# Autodesk Inventor assembly: 51111
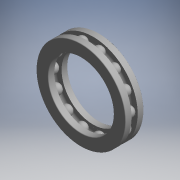
[picture p0: Inventor's stored thumbnail of the model, 180x180]
Saved by Autodesk Inventor 2023 (Build 270158000, 158)
## iProperties
Part Number: 51111
Catalog Web Link: www.cadenas.de
Description: Single Direction Type-
Vendor: NTN
Document SubType Name: Assembly
Designer: partserver
Manufacturer: NTN
Mass: 26.0815 g
Surface Area: 175.483 cm^2
Volume: 26.0815 cm^3
Density: 1 g/cm^3
Category: PARTsolutions
Company: NTN
PSOL_IDENT_0: {$CADENAS_DATA\23d-libs\ntn\ball_roller_bearings\thrust_b\tb_sdt_asmtab.prj},182 {VTYP=3D},{STYP=ASS
PSOL_IDENT_1: TAB},{NB=51111},{LINA=51111},{NN=Single Direction Type},{DATE=21.12.2021 04:23:12},{GEOMDATE=17.04.2
PSOL_IDENT_2: 020 05:29:34},{VERSION=},{LINEID=11140},{WBVAR=},{WBNUMERIC=}  {NB=51111},{LINA=51111},{KT=DUMMY},{I
PSOL_IDENT_3: DNR=},{SD=55},{D=78},{T=16},{R=0.6},{ORDER=51111},{CA=35},{COA=93},{CU=4.2},{CAF=3 550},{COAF=9 500}
PSOL_IDENT_4: ,{NG=2 800},{NO=4 000},{D1=78},{SD1=57},{MASS=0.23},{DA1=69},{DA=64},{RAS=0,6},{X=10.50000},{BN=13.3
PSOL_IDENT_5: 16964},{X1=11.50000},{O=208.81},{T1=5.33333},{T2=5.33333},{RB=4.48000},{PPATH=tb_sdt_asmtpl.prj}
NB: 51111
NN: Single Direction Type
NBSYN: $ORDER.
LINA: 51111
CATALOG: NTN Corporation
SD: 55
D: 78
T: 16
R: 0.6
ORDER: 51111
CA: 35
COA: 93
CU: 4.2
NG: 2 800
NO: 4 000
D1: 78
SD1: 57
MASS: 0.23
SUPPLIER: NTN
ARTICLENO: 51111
BOMINFO: 51111
CREATOR: CADENAS GmbH
Title: 51111
Author: Cadenas PARTsolutions
## Documents named in this file (4)
- C:\Users\adash\OneDrive - Kyushu University\Attachments\ロボコン\catchrobo2022\CAD\Adachi\theta\51111.iam
- C:\Users\adash\OneDrive - Kyushu University\Attachments\ロボコン\catchrobo2022\CAD\Adachi\theta\51111 Housing raceway disc.ipt
- C:\Users\adash\OneDrive - Kyushu University\Attachments\ロボコン\catchrobo2022\CAD\Adachi\theta\51111 Shaft raceway disc.ipt
- C:\Users\adash\OneDrive - Kyushu University\Attachments\ロボコン\catchrobo2022\CAD\Adachi\theta\51111 Ball.ipt
## Components (16 placed, 3 different names)
1. 51111 Housing raceway disc:1 — tb_sdt_hrd_XY@1 <-> tb_sdt_srd_XY@2, tb_sdt_hrd_Z@1 <-> tb_sdt_srd_Z@2, tb_sdt_hrd_YZ@1 <-> tb_sdt_srd_YZ@2
2. 51111 Shaft raceway disc:1 — tb_sdt_hrd_XY@1 <-> tb_sdt_srd_XY@2, tb_sdt_hrd_Z@1 <-> tb_sdt_srd_Z@2, tb_sdt_hrd_YZ@1 <-> tb_sdt_srd_YZ@2, tb_sdt_srd1_1_XY@2 <-> tb_sdt_b_XY@3, tb_sdt_srd1_1_Z@2 <-> tb_sdt_b_Z@3, tb_sdt_srd1_1_YZ@2 <-> tb_sdt_b_YZ@3, tb_sdt_srd1_2_XY@2 <-> tb_sdt_b_XY@4, tb_sdt_srd1_2_Z@2 <-> tb_sdt_b_Z@4, tb_sdt_srd1_2_YZ@2 <-> tb_sdt_b_YZ@4, tb_sdt_srd1_3_XY@2 <-> tb_sdt_b_XY@5, tb_sdt_srd1_3_Z@2 <-> tb_sdt_b_Z@5, tb_sdt_srd1_3_YZ@2 <-> tb_sdt_b_YZ@5, tb_sdt_srd1_4_XY@2 <-> tb_sdt_b_XY@6, tb_sdt_srd1_4_Z@2 <-> tb_sdt_b_Z@6, tb_sdt_srd1_4_YZ@2 <-> tb_sdt_b_YZ@6, tb_sdt_srd1_5_XY@2 <-> tb_sdt_b_XY@7, tb_sdt_srd1_5_Z@2 <-> tb_sdt_b_Z@7, tb_sdt_srd1_5_YZ@2 <-> tb_sdt_b_YZ@7, tb_sdt_srd1_6_XY@2 <-> tb_sdt_b_XY@8, tb_sdt_srd1_6_Z@2 <-> tb_sdt_b_Z@8, tb_sdt_srd1_6_YZ@2 <-> tb_sdt_b_YZ@8, tb_sdt_srd1_7_XY@2 <-> tb_sdt_b_XY@9, tb_sdt_srd1_7_Z@2 <-> tb_sdt_b_Z@9, tb_sdt_srd1_7_YZ@2 <-> tb_sdt_b_YZ@9, tb_sdt_srd1_8_XY@2 <-> tb_sdt_b_XY@10, tb_sdt_srd1_8_Z@2 <-> tb_sdt_b_Z@10, tb_sdt_srd1_8_YZ@2 <-> tb_sdt_b_YZ@10, tb_sdt_srd1_9_XY@2 <-> tb_sdt_b_XY@11, tb_sdt_srd1_9_Z@2 <-> tb_sdt_b_Z@11, tb_sdt_srd1_9_YZ@2 <-> tb_sdt_b_YZ@11, tb_sdt_srd1_10_XY@2 <-> tb_sdt_b_XY@12, tb_sdt_srd1_10_Z@2 <-> tb_sdt_b_Z@12, tb_sdt_srd1_10_YZ@2 <-> tb_sdt_b_YZ@12, tb_sdt_srd1_11_XY@2 <-> tb_sdt_b_XY@13, tb_sdt_srd1_11_Z@2 <-> tb_sdt_b_Z@13, tb_sdt_srd1_11_YZ@2 <-> tb_sdt_b_YZ@13, tb_sdt_srd1_12_XY@2 <-> tb_sdt_b_XY@14, tb_sdt_srd1_12_Z@2 <-> tb_sdt_b_Z@14, tb_sdt_srd1_12_YZ@2 <-> tb_sdt_b_YZ@14, tb_sdt_srd1_13_XY@2 <-> tb_sdt_b_XY@15, tb_sdt_srd1_13_Z@2 <-> tb_sdt_b_Z@15, tb_sdt_srd1_13_YZ@2 <-> tb_sdt_b_YZ@15, tb_sdt_srd1_14_XY@2 <-> tb_sdt_b_XY@16, tb_sdt_srd1_14_Z@2 <-> tb_sdt_b_Z@16, tb_sdt_srd1_14_YZ@2 <-> tb_sdt_b_YZ@16
3. 51111 Ball:1 — tb_sdt_srd1_1_XY@2 <-> tb_sdt_b_XY@3, tb_sdt_srd1_1_Z@2 <-> tb_sdt_b_Z@3, tb_sdt_srd1_1_YZ@2 <-> tb_sdt_b_YZ@3
4. 51111 Ball:2 — tb_sdt_srd1_2_XY@2 <-> tb_sdt_b_XY@4, tb_sdt_srd1_2_Z@2 <-> tb_sdt_b_Z@4, tb_sdt_srd1_2_YZ@2 <-> tb_sdt_b_YZ@4
5. 51111 Ball:3 — tb_sdt_srd1_3_XY@2 <-> tb_sdt_b_XY@5, tb_sdt_srd1_3_Z@2 <-> tb_sdt_b_Z@5, tb_sdt_srd1_3_YZ@2 <-> tb_sdt_b_YZ@5
6. 51111 Ball:4 — tb_sdt_srd1_4_XY@2 <-> tb_sdt_b_XY@6, tb_sdt_srd1_4_Z@2 <-> tb_sdt_b_Z@6, tb_sdt_srd1_4_YZ@2 <-> tb_sdt_b_YZ@6
7. 51111 Ball:5 — tb_sdt_srd1_5_XY@2 <-> tb_sdt_b_XY@7, tb_sdt_srd1_5_Z@2 <-> tb_sdt_b_Z@7, tb_sdt_srd1_5_YZ@2 <-> tb_sdt_b_YZ@7
8. 51111 Ball:6 — tb_sdt_srd1_6_XY@2 <-> tb_sdt_b_XY@8, tb_sdt_srd1_6_Z@2 <-> tb_sdt_b_Z@8, tb_sdt_srd1_6_YZ@2 <-> tb_sdt_b_YZ@8
9. 51111 Ball:7 — tb_sdt_srd1_7_XY@2 <-> tb_sdt_b_XY@9, tb_sdt_srd1_7_Z@2 <-> tb_sdt_b_Z@9, tb_sdt_srd1_7_YZ@2 <-> tb_sdt_b_YZ@9
10. 51111 Ball:8 — tb_sdt_srd1_8_XY@2 <-> tb_sdt_b_XY@10, tb_sdt_srd1_8_Z@2 <-> tb_sdt_b_Z@10, tb_sdt_srd1_8_YZ@2 <-> tb_sdt_b_YZ@10
11. 51111 Ball:9 — tb_sdt_srd1_9_XY@2 <-> tb_sdt_b_XY@11, tb_sdt_srd1_9_Z@2 <-> tb_sdt_b_Z@11, tb_sdt_srd1_9_YZ@2 <-> tb_sdt_b_YZ@11
12. 51111 Ball:10 — tb_sdt_srd1_10_XY@2 <-> tb_sdt_b_XY@12, tb_sdt_srd1_10_Z@2 <-> tb_sdt_b_Z@12, tb_sdt_srd1_10_YZ@2 <-> tb_sdt_b_YZ@12
13. 51111 Ball:11 — tb_sdt_srd1_11_XY@2 <-> tb_sdt_b_XY@13, tb_sdt_srd1_11_Z@2 <-> tb_sdt_b_Z@13, tb_sdt_srd1_11_YZ@2 <-> tb_sdt_b_YZ@13
14. 51111 Ball:12 — tb_sdt_srd1_12_XY@2 <-> tb_sdt_b_XY@14, tb_sdt_srd1_12_Z@2 <-> tb_sdt_b_Z@14, tb_sdt_srd1_12_YZ@2 <-> tb_sdt_b_YZ@14
15. 51111 Ball:13 — tb_sdt_srd1_13_XY@2 <-> tb_sdt_b_XY@15, tb_sdt_srd1_13_Z@2 <-> tb_sdt_b_Z@15, tb_sdt_srd1_13_YZ@2 <-> tb_sdt_b_YZ@15
16. 51111 Ball:14 — tb_sdt_srd1_14_XY@2 <-> tb_sdt_b_XY@16, tb_sdt_srd1_14_Z@2 <-> tb_sdt_b_Z@16, tb_sdt_srd1_14_YZ@2 <-> tb_sdt_b_YZ@16
## Relationships (45: Mate 29, Angle 15, Flush 1)
- tb_sdt_hrd_XY@1 <-> tb_sdt_srd_XY@2 [Flush]: 51111 Housing raceway disc:1 ↔ 51111 Shaft raceway disc:1
- tb_sdt_hrd_Z@1 <-> tb_sdt_srd_Z@2 [Mate]: 51111 Housing raceway disc:1 ↔ 51111 Shaft raceway disc:1
- tb_sdt_hrd_YZ@1 <-> tb_sdt_srd_YZ@2 [Angle] (90 deg): 51111 Housing raceway disc:1 ↔ 51111 Shaft raceway disc:1
- tb_sdt_srd1_1_XY@2 <-> tb_sdt_b_XY@3 [Mate]: 51111 Shaft raceway disc:1 ↔ 51111 Ball:1
- tb_sdt_srd1_1_Z@2 <-> tb_sdt_b_Z@3 [Mate]: 51111 Shaft raceway disc:1 ↔ 51111 Ball:1
- tb_sdt_srd1_1_YZ@2 <-> tb_sdt_b_YZ@3 [Angle] (0 deg): 51111 Shaft raceway disc:1 ↔ 51111 Ball:1
- tb_sdt_srd1_2_XY@2 <-> tb_sdt_b_XY@4 [Mate]: 51111 Shaft raceway disc:1 ↔ 51111 Ball:2
- tb_sdt_srd1_2_Z@2 <-> tb_sdt_b_Z@4 [Mate]: 51111 Shaft raceway disc:1 ↔ 51111 Ball:2
- tb_sdt_srd1_2_YZ@2 <-> tb_sdt_b_YZ@4 [Angle] (0 deg): 51111 Shaft raceway disc:1 ↔ 51111 Ball:2
- tb_sdt_srd1_3_XY@2 <-> tb_sdt_b_XY@5 [Mate]: 51111 Shaft raceway disc:1 ↔ 51111 Ball:3
- tb_sdt_srd1_3_Z@2 <-> tb_sdt_b_Z@5 [Mate]: 51111 Shaft raceway disc:1 ↔ 51111 Ball:3
- tb_sdt_srd1_3_YZ@2 <-> tb_sdt_b_YZ@5 [Angle] (0 deg): 51111 Shaft raceway disc:1 ↔ 51111 Ball:3
- tb_sdt_srd1_4_XY@2 <-> tb_sdt_b_XY@6 [Mate]: 51111 Shaft raceway disc:1 ↔ 51111 Ball:4
- tb_sdt_srd1_4_Z@2 <-> tb_sdt_b_Z@6 [Mate]: 51111 Shaft raceway disc:1 ↔ 51111 Ball:4
- tb_sdt_srd1_4_YZ@2 <-> tb_sdt_b_YZ@6 [Angle] (0 deg): 51111 Shaft raceway disc:1 ↔ 51111 Ball:4
- tb_sdt_srd1_5_XY@2 <-> tb_sdt_b_XY@7 [Mate]: 51111 Shaft raceway disc:1 ↔ 51111 Ball:5
- tb_sdt_srd1_5_Z@2 <-> tb_sdt_b_Z@7 [Mate]: 51111 Shaft raceway disc:1 ↔ 51111 Ball:5
- tb_sdt_srd1_5_YZ@2 <-> tb_sdt_b_YZ@7 [Angle] (0 deg): 51111 Shaft raceway disc:1 ↔ 51111 Ball:5
- tb_sdt_srd1_6_XY@2 <-> tb_sdt_b_XY@8 [Mate]: 51111 Shaft raceway disc:1 ↔ 51111 Ball:6
- tb_sdt_srd1_6_Z@2 <-> tb_sdt_b_Z@8 [Mate]: 51111 Shaft raceway disc:1 ↔ 51111 Ball:6
- tb_sdt_srd1_6_YZ@2 <-> tb_sdt_b_YZ@8 [Angle] (0 deg): 51111 Shaft raceway disc:1 ↔ 51111 Ball:6
- tb_sdt_srd1_7_XY@2 <-> tb_sdt_b_XY@9 [Mate]: 51111 Shaft raceway disc:1 ↔ 51111 Ball:7
- tb_sdt_srd1_7_Z@2 <-> tb_sdt_b_Z@9 [Mate]: 51111 Shaft raceway disc:1 ↔ 51111 Ball:7
- tb_sdt_srd1_7_YZ@2 <-> tb_sdt_b_YZ@9 [Angle] (0 deg): 51111 Shaft raceway disc:1 ↔ 51111 Ball:7
- tb_sdt_srd1_8_XY@2 <-> tb_sdt_b_XY@10 [Mate]: 51111 Shaft raceway disc:1 ↔ 51111 Ball:8
- tb_sdt_srd1_8_Z@2 <-> tb_sdt_b_Z@10 [Mate]: 51111 Shaft raceway disc:1 ↔ 51111 Ball:8
- tb_sdt_srd1_8_YZ@2 <-> tb_sdt_b_YZ@10 [Angle] (0 deg): 51111 Shaft raceway disc:1 ↔ 51111 Ball:8
- tb_sdt_srd1_9_XY@2 <-> tb_sdt_b_XY@11 [Mate]: 51111 Shaft raceway disc:1 ↔ 51111 Ball:9
- tb_sdt_srd1_9_Z@2 <-> tb_sdt_b_Z@11 [Mate]: 51111 Shaft raceway disc:1 ↔ 51111 Ball:9
- tb_sdt_srd1_9_YZ@2 <-> tb_sdt_b_YZ@11 [Angle] (0 deg): 51111 Shaft raceway disc:1 ↔ 51111 Ball:9
- tb_sdt_srd1_10_XY@2 <-> tb_sdt_b_XY@12 [Mate]: 51111 Shaft raceway disc:1 ↔ 51111 Ball:10
- tb_sdt_srd1_10_Z@2 <-> tb_sdt_b_Z@12 [Mate]: 51111 Shaft raceway disc:1 ↔ 51111 Ball:10
- tb_sdt_srd1_10_YZ@2 <-> tb_sdt_b_YZ@12 [Angle] (0 deg): 51111 Shaft raceway disc:1 ↔ 51111 Ball:10
- tb_sdt_srd1_11_XY@2 <-> tb_sdt_b_XY@13 [Mate]: 51111 Shaft raceway disc:1 ↔ 51111 Ball:11
- tb_sdt_srd1_11_Z@2 <-> tb_sdt_b_Z@13 [Mate]: 51111 Shaft raceway disc:1 ↔ 51111 Ball:11
- tb_sdt_srd1_11_YZ@2 <-> tb_sdt_b_YZ@13 [Angle] (0 deg): 51111 Shaft raceway disc:1 ↔ 51111 Ball:11
- tb_sdt_srd1_12_XY@2 <-> tb_sdt_b_XY@14 [Mate]: 51111 Shaft raceway disc:1 ↔ 51111 Ball:12
- tb_sdt_srd1_12_Z@2 <-> tb_sdt_b_Z@14 [Mate]: 51111 Shaft raceway disc:1 ↔ 51111 Ball:12
- tb_sdt_srd1_12_YZ@2 <-> tb_sdt_b_YZ@14 [Angle] (0 deg): 51111 Shaft raceway disc:1 ↔ 51111 Ball:12
- tb_sdt_srd1_13_XY@2 <-> tb_sdt_b_XY@15 [Mate]: 51111 Shaft raceway disc:1 ↔ 51111 Ball:13
- tb_sdt_srd1_13_Z@2 <-> tb_sdt_b_Z@15 [Mate]: 51111 Shaft raceway disc:1 ↔ 51111 Ball:13
- tb_sdt_srd1_13_YZ@2 <-> tb_sdt_b_YZ@15 [Angle] (0 deg): 51111 Shaft raceway disc:1 ↔ 51111 Ball:13
- tb_sdt_srd1_14_XY@2 <-> tb_sdt_b_XY@16 [Mate]: 51111 Shaft raceway disc:1 ↔ 51111 Ball:14
- tb_sdt_srd1_14_Z@2 <-> tb_sdt_b_Z@16 [Mate]: 51111 Shaft raceway disc:1 ↔ 51111 Ball:14
- tb_sdt_srd1_14_YZ@2 <-> tb_sdt_b_YZ@16 [Angle] (0 deg): 51111 Shaft raceway disc:1 ↔ 51111 Ball:14
